# Autodesk Inventor assembly: elbowassembly
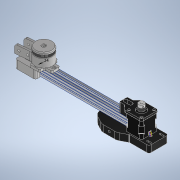
[picture p0: Inventor's stored thumbnail of the model, 180x180]
Saved by Autodesk Inventor 2022 (Build 260153000, 153)
## iProperties
Created: 2022-02-22
Part Number: elbowassembly
Document SubType Name: Assembly
Designer: JK
Author: JK
## Documents named in this file (11)
- C:\Users\JK\Documents\Inventor\ScaraNema\SCARA-3DP\Parts\Elbow\Elbow assembly.iam
- C:\Users\JK\Documents\Inventor\ScaraNema\SCARA-3DP\Parts\Elbow\MOTOR_LONG.ipt
- C:\Users\JK\Documents\Inventor\ScaraNema\SCARA-3DP\Parts\Elbow\RoboDigg GT2 16 pulley.ipt
- C:\Users\JK\Documents\Inventor\ScaraNema\V-Slot 20x20.ipt
- C:\Users\JK\Documents\Inventor\ScaraNema\SCARA-3DP\Parts\Elbow\Elbow motor support.ipt
- C:\Users\JK\Documents\Inventor\ScaraNema\SCARA-3DP\Parts\V-Slot 20x20\V-Slot 20x20-250.ipt
- C:\Users\JK\Documents\Inventor\ScaraNema\SCARA-3DP\Parts\Elbow\Platform.ipt
- C:\Users\JK\Documents\Inventor\ScaraNema\SCARA-3DP\Parts\Elbow\Pulley support.ipt
- C:\Users\JK\Documents\Inventor\ScaraNema\SCARA-3DP\Parts\Elbow\gt264.ipt
- C:\Users\JK\Documents\Inventor\ScaraNema\SCARA-3DP\Parts\Elbow\Tensor.ipt
- C:\Users\JK\Documents\Inventor\ScaraNema\SCARA-3DP\Parts\Elbow\Pulley Top.ipt
## Components (9 placed, 9 different names)
1. MOTOR_LONG:1 — Coincidencia:1, Coincidencia:3, Coincidencia:7, Ángulo:1
2. RoboDigg GT2 16 pulley:1 — Coincidencia:1, Coincidencia:3, Coincidencia:6
3. V-Slot 20x20-250:2 — Coincidencia:8, Ángulo:2, Nivelación:4, Coincidencia:10, Ángulo:3, Coincidencia:13
4. Elbow motor support:1 — Coincidencia:6, Coincidencia:7, Ángulo:1, Coincidencia:9
5. Platform:1 — Coincidencia:8, Ángulo:2, Nivelación:4, Coincidencia:9
6. Pulley support:1 — Coincidencia:10, Ángulo:3, Coincidencia:11, Coincidencia:12, Coincidencia:14
7. gt264:1 — Coincidencia:11, Coincidencia:12, Coincidencia:15, Coincidencia:16
8. Tensor:1 — Coincidencia:13, Coincidencia:14
9. Pulley Top:1 — Coincidencia:15, Coincidencia:16
## Relationships (20: Mate 14, Flush 3, Angle 3)
- Coincidencia:1 [Mate]: MOTOR_LONG:1 ↔ RoboDigg GT2 16 pulley:1
- [Mate]: MOTOR_LONG:1 ↔ V-Slot 20x20-250:2
- [Flush] (10.75 mm): MOTOR_LONG:1 ↔ V-Slot 20x20-250:2
- [Flush]: MOTOR_LONG:1 ↔ V-Slot 20x20-250:2
- Coincidencia:3 [Mate] (3 mm): MOTOR_LONG:1 ↔ RoboDigg GT2 16 pulley:1
- Coincidencia:6 [Mate]: RoboDigg GT2 16 pulley:1 ↔ Elbow motor support:1
- Coincidencia:7 [Mate]: MOTOR_LONG:1 ↔ Elbow motor support:1
- Ángulo:1 [Angle] (0 deg): MOTOR_LONG:1 ↔ Elbow motor support:1
- Coincidencia:8 [Mate]: V-Slot 20x20-250:2 ↔ Platform:1
- Ángulo:2 [Angle] (180 deg): V-Slot 20x20-250:2 ↔ Platform:1
- Nivelación:4 [Flush]: V-Slot 20x20-250:2 ↔ Platform:1
- Coincidencia:9 [Mate]: Elbow motor support:1 ↔ Platform:1
- Coincidencia:10 [Mate]: V-Slot 20x20-250:2 ↔ Pulley support:1
- Ángulo:3 [Angle] (0 deg): V-Slot 20x20-250:2 ↔ Pulley support:1
- Coincidencia:11 [Mate]: Pulley support:1 ↔ gt264:1
- Coincidencia:12 [Mate] (1.8 mm): Pulley support:1 ↔ gt264:1
- Coincidencia:13 [Mate]: V-Slot 20x20-250:2 ↔ Tensor:1
- Coincidencia:14 [Mate]: Pulley support:1 ↔ Tensor:1
- Coincidencia:15 [Mate]: gt264:1 ↔ Pulley Top:1
- Coincidencia:16 [Mate]: gt264:1 ↔ Pulley Top:1
